# Autodesk Inventor assembly: HalfChassisAssem
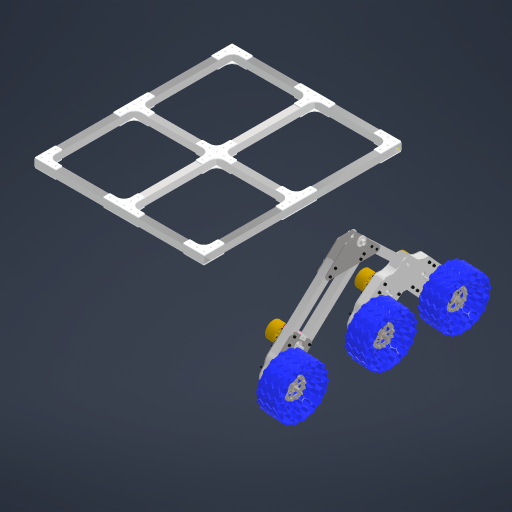
[picture p0: Inventor's stored thumbnail of the model, 512x512]
Saved by Autodesk Inventor 2024 (Build 280153000, 153)
## iProperties
Created: 2023-04-06
Part Number: HalfChassisAssem
Document SubType Name: Assembly
Designer: Dave
Mass: 5362.71 g
Surface Area: 20188.6 cm^2
Volume: 2426.63 cm^3
Density: 2.20995 g/cm^3
Author: Dave
## Documents named in this file (18)
- C:\Users\bugme\OneDrive - The Pennsylvania State University\Documents\GitHub\BehrendURCMechanical\CAD\Chassis V3\HalfChassisAssem.iam
- C:\Users\bugme\OneDrive - The Pennsylvania State University\Documents\GitHub\BehrendURCMechanical\CAD\Chassis V3\L3 Gearbox Assembly.iam
- C:\Users\bugme\OneDrive - The Pennsylvania State University\Documents\GitHub\BehrendURCMechanical\CAD\Chassis V3\L1 Gearbox Assembly.iam
- C:\Users\bugme\OneDrive - The Pennsylvania State University\Documents\GitHub\BehrendURCMechanical\CAD\Chassis V3\HipPivotPlate.ipt
- C:\Users\Dave\Documents\GitHub\BehrendURCMechanical\CAD\Chassis V3\aluminumextrusiontool.ipt
- C:\Users\bugme\OneDrive - The Pennsylvania State University\Documents\GitHub\BehrendURCMechanical\CAD\Chassis V3\aluminumextrusiontool\aluminumextrusiontool-17-10.6in.ipt
- C:\Users\bugme\OneDrive - The Pennsylvania State University\Documents\GitHub\BehrendURCMechanical\CAD\Chassis V3\aluminumextrusiontool\aluminumextrusiontool-17-13.31255in.ipt
- C:\Users\bugme\OneDrive - The Pennsylvania State University\Documents\GitHub\BehrendURCMechanical\CAD\Chassis V3\Pivot Files and Assembly\PivotAssembly.iam
- C:\Users\bugme\OneDrive - The Pennsylvania State University\Documents\GitHub\BehrendURCMechanical\CAD\Chassis V3\aluminumextrusiontool\aluminumextrusiontool-17-7.9.ipt
- C:\Users\bugme\OneDrive - The Pennsylvania State University\Documents\GitHub\BehrendURCMechanical\CAD\Chassis V3\Bolt Nut Washer assem.iam
- C:\Users\bugme\OneDrive - The Pennsylvania State University\Documents\GitHub\BehrendURCMechanical\CAD\Chassis V3\Pivot Files and Assembly\91831A011_18-8 Stainless Steel Nylon-Insert Locknut (1).ipt
- C:\Users\bugme\OneDrive - The Pennsylvania State University\Documents\GitHub\BehrendURCMechanical\CAD\Chassis V3\Wheel\WheelAssembly_v9.iam
- C:\Users\bugme\OneDrive - The Pennsylvania State University\Documents\GitHub\BehrendURCMechanical\CAD\Chassis V3\L3 Gearbox Cover.ipt
- C:\Users\bugme\OneDrive - The Pennsylvania State University\Documents\GitHub\BehrendURCMechanical\CAD\Chassis V3\L1 Gearbox Cover Top.ipt
- C:\Users\bugme\OneDrive - The Pennsylvania State University\Documents\GitHub\BehrendURCMechanical\CAD\Chassis V3\L1 Gearbox Cover.ipt
- C:\Users\bugme\OneDrive - The Pennsylvania State University\Documents\GitHub\BehrendURCMechanical\CAD\Chassis V3\HipCoupler.ipt
- C:\Users\bugme\OneDrive - The Pennsylvania State University\Documents\GitHub\BehrendURCMechanical\CAD\Chassis V3\Body\BodyAssembly.iam
- C:\Users\bugme\OneDrive - The Pennsylvania State University\Documents\GitHub\BehrendURCMechanical\CAD\Chassis V3\aluminumextrusiontool\2.5inTube.ipt
## Components (28 placed, 16 different names)
1. L3 Gearbox Assembly:1 [sub-assembly] — Mate:4, Tangent:2, Mate:10, Insert:1, Mate:14, Mate:15, Mate:16, Mate:17, Mate:18, Mate:19, Mate:20, Mate:56, Mate:57, Mate:58, Mate:59, Mate:60, Mate:61, Mate:62, Mate:63, Mate:64, Mate:65, Mate:66, Mate:67
2. L1 Gearbox Assembly:1 [sub-assembly] — Flush:2, Flush:3, Mate:1, Flush:6, Mate:2, Flush:7, Mate:3, Mate:11, Flush:13, Tangent:3, Mate:12, Mate:13, Flush:14, Mate:21, Mate:22, Mate:24, Mate:25, Mate:26
3. HipPivotPlate:1 — Flush:3, Flush:4, Flush:5, Mate:5, Mate:30, Mate:31, Flush:18, Flush:19, Mate:52, Mate:54
4. HipPivotPlate:2 — Flush:2, Flush:4, Flush:5, Mate:1, Flush:6, Mate:4, Flush:8, Tangent:1, Mate:6, Flush:9, Insert:7, Insert:11, Insert:12, Insert:14, Mate:27, Mate:28, Mate:32, Mate:34, Mate:35, Mate:37, Mate:38, Mate:45, Mate:46, Mate:48, Mate:49, Mate:50, Mate:51, Flush:18, Flush:19, Mate:55
5. aluminumextrusiontool-17-10.6in:1 — Mate:2, Flush:7, Mate:3, Mate:23, Mate:34, Mate:36, Mate:39
6. aluminumextrusiontool-17-7.9:2 — Mate:5, Flush:8, Tangent:1, Tangent:2, Mate:10, Mate:40, Mate:41, Mate:42, Mate:43, Mate:44, Flush:17, Rotation:1, Mate:53
7. aluminumextrusiontool-17-13.31255in:3 — Mate:11, Flush:13, Tangent:3, Flush:17, Mate:52
8. PivotAssembly:2 [sub-assembly] — Insert:1, Insert:16, Rotation:1, Mate:53
9. Bolt Nut Washer assem:1 [sub-assembly] — Insert:7, Mate:37, Mate:38, Mate:39
10. Bolt Nut Washer assem:3 [sub-assembly] — Mate:32, Mate:35, Mate:36
11. Bolt Nut Washer assem:4 [sub-assembly] — Mate:48, Mate:49
12. Bolt Nut Washer assem:5 [sub-assembly] — Insert:11, Mate:50, Mate:51
13. Bolt Nut Washer assem:6 [sub-assembly] — Insert:12, Mate:40, Mate:41, Mate:42, Mate:45
14. Bolt Nut Washer assem:8 [sub-assembly] — Insert:14, Mate:43, Mate:44, Mate:46
15. 91831A011_18-8 Stainless Steel Nylon-Insert Locknut (1):2 — Insert:16
16. WheelAssembly_v9:1 [sub-assembly] — Mate:12, Mate:13, Flush:14, Flush:15
17. WheelAssembly_v9:2 [sub-assembly] — Mate:14, Mate:15, Flush:15, Flush:16
18. WheelAssembly_v9:3 [sub-assembly] — Mate:16, Mate:17, Flush:16
19. L3 Gearbox Cover:1 — Mate:18, Mate:19, Mate:20
20. L1 Gearbox Cover Top:1 — Mate:21, Mate:22, Mate:23
21. L1 Gearbox Cover:1 — Mate:24, Mate:25, Mate:26
22. HipCoupler:1 — Mate:27, Mate:28, Mate:54
23. HipCoupler:2 — Mate:30, Mate:31, Mate:55
24. BodyAssembly:2 [sub-assembly]
25. 2.5inTube:1 — Mate:62, Mate:63, Mate:64
26. 2.5inTube:2 — Mate:65, Mate:66, Mate:67
27. 2.5inTube:3 — Mate:59, Mate:60, Mate:61
28. 2.5inTube:4 — Mate:56, Mate:57, Mate:58
## Relationships (86: Mate 61, Flush 15, Insert 6, Tangent 3, RelateRotation 1)
- Flush:2: L1 Gearbox Assembly:1 ↔ HipPivotPlate:2
- Flush:3: L1 Gearbox Assembly:1 ↔ HipPivotPlate:1
- Flush:4: HipPivotPlate:1 ↔ HipPivotPlate:2
- Flush:5: HipPivotPlate:1 ↔ HipPivotPlate:2
- Mate:1 (396 mm): L1 Gearbox Assembly:1 ↔ HipPivotPlate:2
- Flush:6: L1 Gearbox Assembly:1 ↔ HipPivotPlate:2
- Mate:2: L1 Gearbox Assembly:1 ↔ aluminumextrusiontool-17-10.6in:1
- Flush:7: L1 Gearbox Assembly:1 ↔ aluminumextrusiontool-17-10.6in:1
- Mate:3 (-76.2 mm): L1 Gearbox Assembly:1 ↔ aluminumextrusiontool-17-10.6in:1
- Mate:4 (216 mm): L3 Gearbox Assembly:1 ↔ HipPivotPlate:2
- Mate:5: HipPivotPlate:1 ↔ aluminumextrusiontool-17-7.9:2
- Flush:8: HipPivotPlate:2 ↔ aluminumextrusiontool-17-7.9:2
- Tangent:1 (12.7 mm): HipPivotPlate:2 ↔ aluminumextrusiontool-17-7.9:2
- Tangent:2 (6.35 mm): L3 Gearbox Assembly:1 ↔ aluminumextrusiontool-17-7.9:2
- Mate:6: HipPivotPlate:2
- Flush:9: HipPivotPlate:2
- Mate:10: L3 Gearbox Assembly:1 ↔ aluminumextrusiontool-17-7.9:2
- Mate:11: L1 Gearbox Assembly:1 ↔ aluminumextrusiontool-17-13.31255in:3
- Flush:13: L1 Gearbox Assembly:1 ↔ aluminumextrusiontool-17-13.31255in:3
- Tangent:3 (12.7 mm): L1 Gearbox Assembly:1 ↔ aluminumextrusiontool-17-13.31255in:3
- Insert:1: L3 Gearbox Assembly:1 ↔ PivotAssembly:2
- Insert:7: HipPivotPlate:2 ↔ Bolt Nut Washer assem:1
- Insert:11: HipPivotPlate:2 ↔ Bolt Nut Washer assem:5
- Insert:12: HipPivotPlate:2 ↔ Bolt Nut Washer assem:6
- Insert:14: HipPivotPlate:2 ↔ Bolt Nut Washer assem:8
- Insert:16: PivotAssembly:2 ↔ 91831A011_18-8 Stainless Steel Nylon-Insert Locknut (1):2
- Mate:12: L1 Gearbox Assembly:1 ↔ WheelAssembly_v9:1
- Mate:13: L1 Gearbox Assembly:1 ↔ WheelAssembly_v9:1
- Flush:14 (19.05 mm): L1 Gearbox Assembly:1 ↔ WheelAssembly_v9:1
- Mate:14: L3 Gearbox Assembly:1 ↔ WheelAssembly_v9:2
- Mate:15: L3 Gearbox Assembly:1 ↔ WheelAssembly_v9:2
- Mate:16: L3 Gearbox Assembly:1 ↔ WheelAssembly_v9:3
- Mate:17: L3 Gearbox Assembly:1 ↔ WheelAssembly_v9:3
- Flush:15: WheelAssembly_v9:1 ↔ WheelAssembly_v9:2
- Flush:16: WheelAssembly_v9:2 ↔ WheelAssembly_v9:3
- Mate:18: L3 Gearbox Assembly:1 ↔ L3 Gearbox Cover:1
- Mate:19: L3 Gearbox Assembly:1 ↔ L3 Gearbox Cover:1
- Mate:20: L3 Gearbox Assembly:1 ↔ L3 Gearbox Cover:1
- Mate:21: L1 Gearbox Assembly:1 ↔ L1 Gearbox Cover Top:1
- Mate:22: L1 Gearbox Assembly:1 ↔ L1 Gearbox Cover Top:1
- Mate:23: aluminumextrusiontool-17-10.6in:1 ↔ L1 Gearbox Cover Top:1
- Mate:24: L1 Gearbox Assembly:1 ↔ L1 Gearbox Cover:1
- Mate:25: L1 Gearbox Assembly:1 ↔ L1 Gearbox Cover:1
- Mate:26: L1 Gearbox Assembly:1 ↔ L1 Gearbox Cover:1
- Mate:27: HipPivotPlate:2 ↔ HipCoupler:1
- Mate:28: HipPivotPlate:2 ↔ HipCoupler:1
- Mate:30: HipPivotPlate:1 ↔ HipCoupler:2
- Mate:31: HipPivotPlate:1 ↔ HipCoupler:2
- Mate:32: HipPivotPlate:2 ↔ Bolt Nut Washer assem:3
- Mate:34: HipPivotPlate:2 ↔ aluminumextrusiontool-17-10.6in:1
- Mate:35: HipPivotPlate:2 ↔ Bolt Nut Washer assem:3
- Mate:36: aluminumextrusiontool-17-10.6in:1 ↔ Bolt Nut Washer assem:3
- Mate:37: HipPivotPlate:2 ↔ Bolt Nut Washer assem:1
- Mate:38: HipPivotPlate:2 ↔ Bolt Nut Washer assem:1
- Mate:39: aluminumextrusiontool-17-10.6in:1 ↔ Bolt Nut Washer assem:1
- Mate:40: aluminumextrusiontool-17-7.9:2 ↔ Bolt Nut Washer assem:6
- Mate:41: aluminumextrusiontool-17-7.9:2 ↔ Bolt Nut Washer assem:6
- Mate:42: aluminumextrusiontool-17-7.9:2 ↔ Bolt Nut Washer assem:6
- Mate:43: aluminumextrusiontool-17-7.9:2 ↔ Bolt Nut Washer assem:8
- Mate:44: aluminumextrusiontool-17-7.9:2 ↔ Bolt Nut Washer assem:8
- Mate:45: HipPivotPlate:2 ↔ Bolt Nut Washer assem:6
- Mate:46: HipPivotPlate:2 ↔ Bolt Nut Washer assem:8
- Flush:17: aluminumextrusiontool-17-7.9:2 ↔ aluminumextrusiontool-17-13.31255in:3
- Mate:48: HipPivotPlate:2 ↔ Bolt Nut Washer assem:4
- Mate:49: HipPivotPlate:2 ↔ Bolt Nut Washer assem:4
- Mate:50: HipPivotPlate:2 ↔ Bolt Nut Washer assem:5
- Mate:51: HipPivotPlate:2 ↔ Bolt Nut Washer assem:5
- Flush:18: HipPivotPlate:1 ↔ HipPivotPlate:2
- Flush:19: HipPivotPlate:1 ↔ HipPivotPlate:2
- Mate:52: HipPivotPlate:1 ↔ aluminumextrusiontool-17-13.31255in:3
- Rotation:1 [RelateRotation] (2 ul): aluminumextrusiontool-17-7.9:2 ↔ PivotAssembly:2
- Mate:53: aluminumextrusiontool-17-7.9:2 ↔ PivotAssembly:2
- Mate:54: HipPivotPlate:1 ↔ HipCoupler:1
- Mate:55: HipPivotPlate:2 ↔ HipCoupler:2
- Mate:56: L3 Gearbox Assembly:1 ↔ 2.5inTube:4
- Mate:57: L3 Gearbox Assembly:1 ↔ 2.5inTube:4
- Mate:58: L3 Gearbox Assembly:1 ↔ 2.5inTube:4
- Mate:59: L3 Gearbox Assembly:1 ↔ 2.5inTube:3
- Mate:60: L3 Gearbox Assembly:1 ↔ 2.5inTube:3
- Mate:61: L3 Gearbox Assembly:1 ↔ 2.5inTube:3
- Mate:62: L3 Gearbox Assembly:1 ↔ 2.5inTube:1
- Mate:63: L3 Gearbox Assembly:1 ↔ 2.5inTube:1
- Mate:64: L3 Gearbox Assembly:1 ↔ 2.5inTube:1
- Mate:65: L3 Gearbox Assembly:1 ↔ 2.5inTube:2
- Mate:66: L3 Gearbox Assembly:1 ↔ 2.5inTube:2
- Mate:67: L3 Gearbox Assembly:1 ↔ 2.5inTube:2
